# Autodesk Inventor assembly: Back_Case
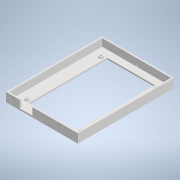
[picture p0: Inventor's stored thumbnail of the model, 180x180]
Saved by Autodesk Inventor 2020.2 (Build 242310000, 310)
## iProperties
Created: 2020-04-06
Part Number: Back_Case
Document SubType Name: Assembly
Designer: Mitch
Author: Mitch
## Documents named in this file (5)
- E:\Youtube Channel\Pojects\Raspberry pi\Raspi Cloud Smart Frame\Mech\Back_Case.iam
- E:\Youtube Channel\Pojects\Raspberry pi\Raspi Cloud Smart Frame\Mech\Dispaly.ipt
- E:\Youtube Channel\Pojects\Raspberry pi\Raspi Cloud Smart Frame\Mech\Inner Case.ipt
- E:\Youtube Channel\Pojects\Raspberry pi\Raspi Cloud Smart Frame\Mech\Vented Case.ipt
- E:\Youtube Channel\Pojects\Raspberry pi\Raspi Cloud Smart Frame\Mech\raspberrypi_3_stripped.iam
## Components (4 placed, 4 different names)
1. Dispaly:1 — Mate:1, Mate:2, Mate:3
2. Inner Case:1 — Mate:1, Mate:2, Mate:3, Mate:7, Mate:8, Flush:1
3. raspberrypi_3_stripped:1 [sub-assembly] — Mate:4, Mate:5, Mate:6
4. Vented Case:2 — Mate:4, Mate:5, Mate:6, Mate:7, Mate:8, Flush:1
## Relationships (9: Mate 8, Flush 1)
- Mate:1: Dispaly:1 ↔ Inner Case:1
- Mate:2: Dispaly:1 ↔ Inner Case:1
- Mate:3: Dispaly:1 ↔ Inner Case:1
- Mate:4 (50.8 mm): raspberrypi_3_stripped:1 ↔ Vented Case:2
- Mate:5 (58.8264 mm): raspberrypi_3_stripped:1 ↔ Vented Case:2
- Mate:6: raspberrypi_3_stripped:1 ↔ Vented Case:2
- Mate:7 (0.254 mm): Inner Case:1 ↔ Vented Case:2
- Mate:8 (0.254 mm): Inner Case:1 ↔ Vented Case:2
- Flush:1 (9.525 mm): Inner Case:1 ↔ Vented Case:2
